# Autodesk Inventor assembly: Узел потенциометра
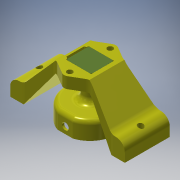
[picture p0: Inventor's stored thumbnail of the model, 180x180]
Saved by Autodesk Inventor 2019.1 (Build 231200000, 200)
## iProperties
Created: 2018-10-15
Part Number: Узел потенциометра
Material: Типовые
Document SubType Name: Assembly
Designer: Олег
Author: Олег
## Documents named in this file (4)
- C:\Users\Олег\OneDrive\Общая\NoSpace 2.0\Манипулятор\Узел потенциометра.iam
- C:\Users\Олег\OneDrive\Общая\NoSpace 2.0\Манипулятор\Переходная шайба между осью и потенциометром.ipt
- C:\Users\Олег\OneDrive\Общая\NoSpace 2.0\Манипулятор\Потенциометр.ipt
- C:\Users\Олег\OneDrive\Общая\NoSpace 2.0\Манипулятор\Фиксатор потенциометра.ipt
## Components (3 placed, 3 different names)
1. Переходная шайба между осью и потенциометром:1 — Совмещение:4, Совмещение:5, Угол:1
2. Потенциометр:1 — Совмещение:1, Совмещение:2, Совмещение:3, Совмещение:4, Совмещение:5
3. Фиксатор потенциометра:1 — Совмещение:1, Совмещение:2, Совмещение:3, Угол:1
## Relationships (6: Mate 5, Angle 1)
- Совмещение:1 [Mate]: Потенциометр:1 ↔ Фиксатор потенциометра:1
- Совмещение:2 [Mate]: Потенциометр:1 ↔ Фиксатор потенциометра:1
- Совмещение:3 [Mate]: Потенциометр:1 ↔ Фиксатор потенциометра:1
- Совмещение:4 [Mate] (1 mm): Переходная шайба между осью и потенциометром:1 ↔ Потенциометр:1
- Совмещение:5 [Mate]: Переходная шайба между осью и потенциометром:1 ↔ Потенциометр:1
- Угол:1 [Angle] (0 deg): Переходная шайба между осью и потенциометром:1 ↔ Фиксатор потенциометра:1
